# Autodesk Inventor assembly: shooter launcher
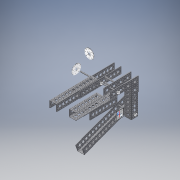
[picture p0: Inventor's stored thumbnail of the model, 180x180]
Saved by Autodesk Inventor 2017 (Build 210142000, 142)
## iProperties
Created: 2018-05-23
Part Number: shooter launcher
Document SubType Name: Assembly
Designer: User
Author: User
## Documents named in this file (12)
- C:\Robotics\CAD\2018-19_CAD\Offseason\shooter launcher.iam
- C:\Robotics\CAD\COTSParts\Actobotics\585 parts\585446Channel6in.ipt
- C:\Robotics\CAD\COTSParts\Actobotics\585 parts\585628FlatPattern90degreesA.ipt
- C:\Robotics\CAD\COTSParts\Tetrix\Hex standoff 2in.ipt
- C:\Robotics\CAD\COTSParts\Actobotics\634 parts\634088.25inDShaft8inLong.ipt
- C:\Robotics\CAD\COTSParts\Actobotics\615 parts\615106Sprocket.5inBore.25inPitch24Teeth.ipt
- C:\Robotics\CAD\COTSParts\Actobotics\535 parts\535198Bearing.25ID.5OD.ipt
- C:\Robotics\CAD\COTSParts\Actobotics\Collar.ipt
- C:\Robotics\CAD\COTSParts\Actobotics\585 parts\585450Channel9in.ipt
- C:\Robotics\CAD\COTSParts\Actobotics\585 parts\585454Channel12in.ipt
- C:\Robotics\CAD\COTSParts\Actobotics\634 parts\634080.25inDShaft4inLong.ipt
- C:\Robotics\CAD\COTSParts\Fasteners\Nylon spacer .25.ipt
## Components (30 placed, 11 different names)
1. 585446Channel6in:1 — Mate:1, Flush:1, Flush:2, Mate:2, Flush:4, Mate:3, Flush:6, Insert:1, Insert:4, Mate:10, Mate:11, Mate:12, Mate:13, Mate:14, Insert:9, Flush:7, Insert:11
2. 585446Channel6in:2 — Mate:1, Flush:1, Flush:2, Flush:3, Flush:5, Mate:26, Mate:27, Mate:28, Mate:29
3. 585628FlatPattern90degreesA:1 — Mate:3, Flush:5, Flush:6
4. 585628FlatPattern90degreesA:2 — Mate:2, Flush:3, Flush:4
5. Hex standoff 2in:1 — Insert:11
6. Hex standoff 2in:3 — Insert:1, Mate:25
7. 634088.25inDShaft8inLong:1 — Insert:4, Mate:5, Angle:1, Angle:2, Angle:3, Angle:4, Mate:22
8. 615106Sprocket.5inBore.25inPitch24Teeth:1 — Mate:5
9. 615106Sprocket.5inBore.25inPitch24Teeth:2
10. 535198Bearing.25ID.5OD:1 — Insert:10, Mate:21
11. 535198Bearing.25ID.5OD:2 — Mate:12, Mate:13, Insert:5
12. 535198Bearing.25ID.5OD:3 — Mate:10, Mate:11, Insert:6
13. 535198Bearing.25ID.5OD:4 — Insert:8, Mate:22, Mate:23
14. Collar:1 — Angle:2, Insert:6, Mate:20
15. Collar:2 — Insert:5, Angle:1
16. Collar:3 — Angle:3, Mate:21
17. Collar:4 — Insert:8, Angle:4
18. 585446Channel6in:3 — Mate:14, Insert:9, Flush:7, Mate:15, Flush:8, Mate:16
19. 585446Channel6in:4 — Mate:15, Flush:8, Mate:16, Flush:9
20. 585450Channel9in:1 — Mate:17, Mate:19, Mate:20, Insert:10, Mate:23, Flush:9, Mate:24, Mate:25
21. 585450Channel9in:2 — Mate:17, Mate:19, Mate:24
22. 585454Channel12in:1 — Mate:30, Mate:31, Mate:36, Mate:37, Mate:38
23. 634080.25inDShaft4inLong:1 — Mate:39, Mate:40, Mate:44, Mate:46
24. 535198Bearing.25ID.5OD:5 — Mate:36, Mate:37, Mate:38, Mate:43
25. 535198Bearing.25ID.5OD:6 — Mate:28, Mate:29, Mate:41
26. 535198Bearing.25ID.5OD:7 — Mate:30, Mate:31, Mate:40, Mate:45
27. 535198Bearing.25ID.5OD:8 — Mate:26, Mate:27, Mate:34, Mate:35
28. Collar:5 — Mate:34, Mate:35, Mate:39
29. Collar:6 — Mate:43, Mate:44
30. Nylon spacer .25:1 — Mate:41, Mate:45, Mate:46
## Relationships (58: Mate 37, Flush 9, Insert 8, Angle 4)
- Mate:1: 585446Channel6in:1 ↔ 585446Channel6in:2
- Flush:1: 585446Channel6in:1 ↔ 585446Channel6in:2
- Flush:2: 585446Channel6in:1 ↔ 585446Channel6in:2
- Mate:2: 585446Channel6in:1 ↔ 585628FlatPattern90degreesA:2
- Flush:3: 585446Channel6in:2 ↔ 585628FlatPattern90degreesA:2
- Flush:4: 585446Channel6in:1 ↔ 585628FlatPattern90degreesA:2
- Mate:3: 585446Channel6in:1 ↔ 585628FlatPattern90degreesA:1
- Flush:5: 585446Channel6in:2 ↔ 585628FlatPattern90degreesA:1
- Flush:6: 585446Channel6in:1 ↔ 585628FlatPattern90degreesA:1
- Insert:1: 585446Channel6in:1 ↔ Hex standoff 2in:3
- Insert:4 (7.1882 mm): 585446Channel6in:1 ↔ 634088.25inDShaft8inLong:1
- Mate:5: 634088.25inDShaft8inLong:1 ↔ 615106Sprocket.5inBore.25inPitch24Teeth:1
- Mate:10: 585446Channel6in:1 ↔ 535198Bearing.25ID.5OD:3
- Mate:11: 585446Channel6in:1 ↔ 535198Bearing.25ID.5OD:3
- Mate:12: 585446Channel6in:1 ↔ 535198Bearing.25ID.5OD:2
- Mate:13: 585446Channel6in:1 ↔ 535198Bearing.25ID.5OD:2
- Insert:5: 535198Bearing.25ID.5OD:2 ↔ Collar:2
- Angle:1 (0 deg): 634088.25inDShaft8inLong:1 ↔ Collar:2
- Angle:2 (0 deg): 634088.25inDShaft8inLong:1 ↔ Collar:1
- Insert:6: 535198Bearing.25ID.5OD:3 ↔ Collar:1
- Angle:3 (0 deg): 634088.25inDShaft8inLong:1 ↔ Collar:3
- Insert:8: 535198Bearing.25ID.5OD:4 ↔ Collar:4
- Angle:4 (0 deg): 634088.25inDShaft8inLong:1 ↔ Collar:4
- Mate:14: 585446Channel6in:1 ↔ 585446Channel6in:3
- Insert:9: 585446Channel6in:1 ↔ 585446Channel6in:3
- Flush:7: 585446Channel6in:1 ↔ 585446Channel6in:3
- Mate:15: 585446Channel6in:3 ↔ 585446Channel6in:4
- Flush:8: 585446Channel6in:3 ↔ 585446Channel6in:4
- Mate:16: 585446Channel6in:3 ↔ 585446Channel6in:4
- Mate:17: 585450Channel9in:1 ↔ 585450Channel9in:2
- Mate:19 (-101.6 mm): 585450Channel9in:1 ↔ 585450Channel9in:2
- Mate:20: Collar:1 ↔ 585450Channel9in:1
- Insert:10: 535198Bearing.25ID.5OD:1 ↔ 585450Channel9in:1
- Mate:21: 535198Bearing.25ID.5OD:1 ↔ Collar:3
- Mate:22: 634088.25inDShaft8inLong:1 ↔ 535198Bearing.25ID.5OD:4
- Mate:23: 535198Bearing.25ID.5OD:4 ↔ 585450Channel9in:1
- Flush:9: 585446Channel6in:4 ↔ 585450Channel9in:1
- Mate:24: 585450Channel9in:1 ↔ 585450Channel9in:2
- Insert:11: 585446Channel6in:1 ↔ Hex standoff 2in:1
- Mate:25: Hex standoff 2in:3 ↔ 585450Channel9in:1
- Mate:26: 585446Channel6in:2 ↔ 535198Bearing.25ID.5OD:8
- Mate:27: 585446Channel6in:2 ↔ 535198Bearing.25ID.5OD:8
- Mate:28: 585446Channel6in:2 ↔ 535198Bearing.25ID.5OD:6
- Mate:29: 585446Channel6in:2 ↔ 535198Bearing.25ID.5OD:6
- Mate:30: 585454Channel12in:1 ↔ 535198Bearing.25ID.5OD:7
- Mate:31: 585454Channel12in:1 ↔ 535198Bearing.25ID.5OD:7
- Mate:34: 535198Bearing.25ID.5OD:8 ↔ Collar:5
- Mate:35: 535198Bearing.25ID.5OD:8 ↔ Collar:5
- Mate:36: 585454Channel12in:1 ↔ 535198Bearing.25ID.5OD:5
- Mate:37: 585454Channel12in:1 ↔ 535198Bearing.25ID.5OD:5
- Mate:38: 585454Channel12in:1 ↔ 535198Bearing.25ID.5OD:5
- Mate:39: 634080.25inDShaft4inLong:1 ↔ Collar:5
- Mate:40: 634080.25inDShaft4inLong:1 ↔ 535198Bearing.25ID.5OD:7
- Mate:41: 535198Bearing.25ID.5OD:6 ↔ Nylon spacer .25:1
- Mate:43: 535198Bearing.25ID.5OD:5 ↔ Collar:6
- Mate:44: 634080.25inDShaft4inLong:1 ↔ Collar:6
- Mate:45: 535198Bearing.25ID.5OD:7 ↔ Nylon spacer .25:1
- Mate:46: 634080.25inDShaft4inLong:1 ↔ Nylon spacer .25:1
